# Autodesk Inventor assembly: Placek
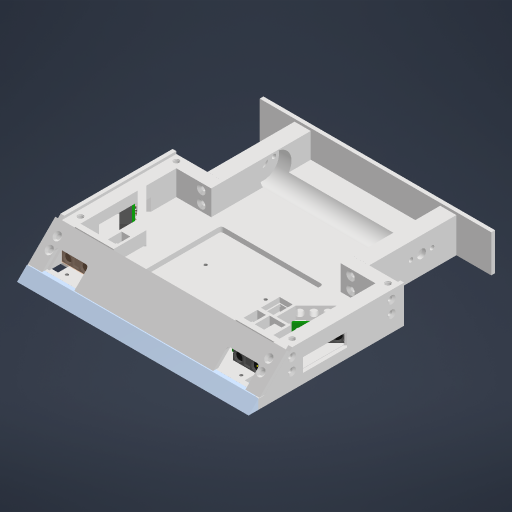
[picture p0: Inventor's stored thumbnail of the model, 512x512]
Saved by Autodesk Inventor 2023 (Build 270158000, 158)
## iProperties
Created: 2023-03-15
Part Number: Placek
Document SubType Name: Assembly
Designer: Michał
Author: Michał
## Documents named in this file (12)
- D:\Projekty\RoboIlo\Placek\3D\Placek.iam
- D:\Projekty\RoboIlo\Placek\3D\blacha.ipt
- D:\Projekty\RoboIlo\Placek\3D\mocowanie silnika.ipt
- D:\Projekty\RoboIlo\Placek\3D\mocowanie silnika_MIR.ipt
- D:\Projekty\RoboIlo\Placek\3D\mocowanie-czujniklewy.ipt
- D:\Projekty\RoboIlo\Placek\3D\PLUG.ipt
- D:\Projekty\RoboIlo\Placek\3D\tyl.ipt
- D:\Projekty\RoboIlo\Placek\3D\BokPrawy.ipt
- D:\Projekty\RoboIlo\Placek\3D\sds02a-with-sensor.ipt
- D:\Projekty\RoboIlo\Placek\3D\mocowanie-czujnika-p.ipt
- D:\Projekty\RoboIlo\Placek\3D\BokPrawy_MIR.ipt
- D:\Projekty\RoboIlo\Placek\3D\Przod.ipt
## Components (14 placed, 11 different names)
1. blacha:1 — Insert:1, Insert:2, Insert:3, Insert:4, Insert:5, Insert:6, Insert:8, Insert:9, Insert:16, Insert:17, Angle:3, Angle:4
2. mocowanie silnika:1 — Insert:5, Insert:6, Insert:10
3. mocowanie silnika_MIR:1 — Insert:3, Insert:4, Insert:11
4. mocowanie-czujniklewy:1 — Insert:8, Insert:9, Insert:14, Insert:15, Angle:2
5. PLUG:1 — Insert:1, Insert:2, Mate:1, Mate:2
6. tyl:1 — Insert:10, Insert:11, Mate:3
7. BokPrawy:1 — Flush:1, Flush:2
8. sds02a-with-sensor:1 — Insert:19, Angle:1, Flush:3
9. sds02a-with-sensor:2 — Insert:18, Angle:4, Flush:1
10. sds02a-with-sensor:3 — Insert:15, Angle:3
11. sds02a-with-sensor:4 — Insert:14, Angle:2
12. mocowanie-czujnika-p:1 — Insert:16, Insert:17, Insert:18, Insert:19, Angle:1
13. BokPrawy_MIR:1
14. Przod:1 — Flush:2, Flush:3
## Relationships (26: Insert 16, Angle 4, Flush 3, Mate 3)
- Insert:1: blacha:1 ↔ PLUG:1
- Insert:2: blacha:1 ↔ PLUG:1
- Insert:3: blacha:1 ↔ mocowanie silnika_MIR:1
- Insert:4: blacha:1 ↔ mocowanie silnika_MIR:1
- Insert:5: blacha:1 ↔ mocowanie silnika:1
- Insert:6: blacha:1 ↔ mocowanie silnika:1
- Insert:8: blacha:1 ↔ mocowanie-czujniklewy:1
- Insert:9: blacha:1 ↔ mocowanie-czujniklewy:1
- Insert:10: mocowanie silnika:1 ↔ tyl:1
- Insert:11: mocowanie silnika_MIR:1 ↔ tyl:1
- Insert:14: mocowanie-czujniklewy:1 ↔ sds02a-with-sensor:4
- Insert:15: mocowanie-czujniklewy:1 ↔ sds02a-with-sensor:3
- Insert:16: blacha:1 ↔ mocowanie-czujnika-p:1
- Insert:17: blacha:1 ↔ mocowanie-czujnika-p:1
- Insert:18: sds02a-with-sensor:2 ↔ mocowanie-czujnika-p:1
- Insert:19: sds02a-with-sensor:1 ↔ mocowanie-czujnika-p:1
- Angle:1 (0 deg): sds02a-with-sensor:1 ↔ mocowanie-czujnika-p:1
- Angle:2 (0 deg): mocowanie-czujniklewy:1 ↔ sds02a-with-sensor:4
- Angle:3 (0 deg): blacha:1 ↔ sds02a-with-sensor:3
- Angle:4 (0 deg): blacha:1 ↔ sds02a-with-sensor:2
- Flush:1: BokPrawy:1 ↔ sds02a-with-sensor:2
- Mate:1: PLUG:1
- Mate:2: PLUG:1
- Mate:3: tyl:1
- Flush:2: BokPrawy:1 ↔ Przod:1
- Flush:3: sds02a-with-sensor:1 ↔ Przod:1
